# Autodesk Inventor assembly: Bottom Roller
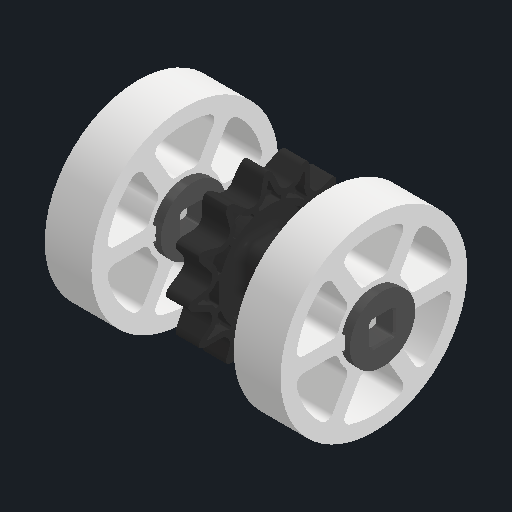
[picture p0: Inventor's stored thumbnail of the model, 512x512]
Saved by Autodesk Inventor 2025 (Build 290162000, 162)
## iProperties
Created: 2024-12-25
Part Number: Bottom Roller
Document SubType Name: Assembly
Designer: Averey Ku
Author: Averey Ku
## Documents named in this file (4)
- D:\VEX\High Stakes\CAD\V4\Conveyer\Bottom Roller.iam
- D:\VEX\High Stakes\CAD\ROBOPROS-CAD-Inventor\Motion\Sprockets\9P Sprocket\9P 12T Sprocket, No Insert.iam
- D:\VEX\High Stakes\CAD\ROBOPROS-CAD-Inventor\Motion\Sprockets\9P Sprocket.iam
- D:\VEX\High Stakes\CAD\ROBOPROS-CAD-Inventor\Quick Assemblies\2.000 30A .500 With Adapters.iam
## Components (3 placed, 2 different names)
1. 9P 12T Sprocket, No Insert:1 [sub-assembly] — Insert:1, Insert:2
2. 2.000 30A .500 With Adapters:1 [sub-assembly] — Insert:1
3. 2.000 30A .500 With Adapters:2 [sub-assembly] — Insert:2
## Relationships (2: Insert 2)
- Insert:1 (10.3188 mm): 9P 12T Sprocket, No Insert:1 ↔ 2.000 30A .500 With Adapters:1
- Insert:2 (10.3188 mm): 9P 12T Sprocket, No Insert:1 ↔ 2.000 30A .500 With Adapters:2
